# Autodesk Inventor assembly: ConceleadHinges
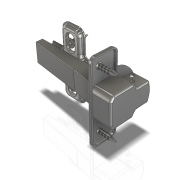
[picture p0: Inventor's stored thumbnail of the model, 180x180]
Saved by Autodesk Inventor 2024 (Build 280153000, 153)
## iProperties
RuleStatus: InUse
Created: 2023-02-09
Part Number: ConceleadHinges
Document SubType Name: Assembly
Designer: sauliusd
Author: sauliusd
## Documents named in this file (4)
- C:\W4INV 2024 Design\SMART HARDWARE\Concelead Hinges\ConceleadHinges.iam
- C:\W4INV 2024 Design\SMART HARDWARE\Concelead Hinges\Parts\Concelead Hinges Skeleton.ipt
- C:\W4INV 2024 Design\LIBRARY\Hinges\CONCEALED HINGE\Inset Hinge Wood Screw Cup Wood Screw T18.iam
- C:\W4INV 2023 Design\LIBRARY\Hinges\CONCEALED HINGE.iam
## Components (3 placed, 3 different names)
1. @Skeleton — Overlay Carcass Flush, Overlay Axis Flush, Overlay Door Flush, Inset Door Flush, Inset Carcass Flush, Inset Axis Flush
2. ConceleadHinge [sub-assembly] — Overlay Carcass Flush, Overlay Axis Flush, Overlay Door Flush, Inset Door Flush, Inset Carcass Flush, Inset Axis Flush
3. Inset Hinge Wood Screw Cup Wood Screw T18:2 [sub-assembly]
## Component patterns: (2 elements, first: ConceleadHinge)
## Relationships (6: Flush 5, Mate 1)
- Overlay Carcass Flush [Flush]: @Skeleton ↔ ConceleadHinge
- Overlay Axis Flush [Flush]: @Skeleton ↔ ConceleadHinge
- Overlay Door Flush [Flush]: @Skeleton ↔ ConceleadHinge
- Inset Door Flush [Flush]: @Skeleton ↔ ConceleadHinge
- Inset Carcass Flush [Flush]: @Skeleton ↔ ConceleadHinge
- Inset Axis Flush [Mate]: @Skeleton ↔ ConceleadHinge
## Named parameters: HingesNumber = 2, OffsetFromSidePlusSide = 60 mm, OffsetFromSideMinusSide = 60 mm, ContactPatchWidth = 600 mm, ContactPatchHeight = 18 mm, NestledBoardT = 18 mm, PillarBoardT = 18 mm, ContactAngle = 90 deg, Gap = 2 mm
